# Autodesk Inventor assembly: Alternative Pump Assembley
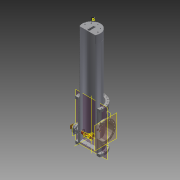
[picture p0: Inventor's stored thumbnail of the model, 180x180]
Saved by Autodesk Inventor 2015 (Build 190159000, 159)
## iProperties
Created: 2014-05-21
Part Number: Alternative Pump Assembley
Document SubType Name: Assembly
Designer: jad211
Author: jad211
## Documents named in this file (5)
- C:\CADFiles\EDM Machine\EDM New Pumping Region\Alternative Pump Assembley.iam
- C:\CADFiles\EDM Machine\EDM Beamline\Chamber parts\hudson chamber actual size.ipt
- C:\CADFiles\EDM Machine\EDM Inner Shield\Inner Shield.iam
- C:\CADFiles\EDM Machine\EDM New Pumping Region\table.ipt
- C:\CADFiles\EDM Machine\EDM New Pumping Region\microwave rf pump region.iam
## Components (4 placed, 4 different names)
1. hudson chamber actual size:1 — Mate:1, Mate:2, Mate:3
2. Inner Shield:1 [sub-assembly] — Mate:3, Mate:4, Flush:1, Mate:9, Mate:10
3. table:1 — Flush:1, Mate:9, Mate:10
4. microwave rf pump region:1 [sub-assembly] — Mate:11, Mate:12, Mate:13
## Relationships (10: Mate 9, Flush 1)
- Mate:1: hudson chamber actual size:1
- Mate:2: hudson chamber actual size:1
- Mate:3: hudson chamber actual size:1 ↔ Inner Shield:1
- Mate:4: Inner Shield:1
- Flush:1: Inner Shield:1 ↔ table:1
- Mate:9: Inner Shield:1 ↔ table:1
- Mate:10: Inner Shield:1 ↔ table:1
- Mate:11: microwave rf pump region:1
- Mate:12: microwave rf pump region:1
- Mate:13: microwave rf pump region:1
